# Autodesk Inventor assembly: лимонадный автомат
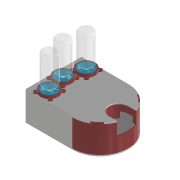
[picture p0: Inventor's stored thumbnail of the model, 180x180]
Saved by Autodesk Inventor 2022 (Build 260153000, 153)
## iProperties
Created: 2025-01-24
Part Number: лимонадный автомат
Document SubType Name: Assembly
Designer: Ivan
Author: Ivan
## Documents named in this file (8)
- E:\ВСЕ ДЕТАЛИ\лимонадный автомат.iam
- Лимонадный автомат_.iam
- E:\shoter4\Корпус.iam
- E:\shoter4\Основание верхнее.ipt
- E:\shoter4\Поворотный_модуль.iam
- E:\shoter4\Pump_V4.iam
- E:\shoter4\Держатель.ipt
- E:\ВСЕ ДЕТАЛИ\узел бутылки.iam
## Components (12 placed, 6 different names)
1. Корпус:1 [sub-assembly] — Совмещение:1, Заподлицо:1, Заподлицо:2, Совмещение:2, Совмещение:12, Совмещение:13, Совмещение:22, Совмещение:23, Совмещение:24, Совмещение:25, Совмещение:26, Совмещение:27, Совмещение:30, Совмещение:31, Совмещение:32
2. Основание верхнее:1 — Совмещение:1, Заподлицо:1, Заподлицо:2, Совмещение:2, Совмещение:33, Совмещение:34, Совмещение:35, Совмещение:36, Совмещение:37, Совмещение:38
3. Поворотный_модуль:1 [sub-assembly] — Совмещение:12, Совмещение:13
4. Pump_V4:3 [sub-assembly] — Заподлицо:5, Совмещение:18, Совмещение:19
5. Pump_V4:4 [sub-assembly] — Заподлицо:6, Совмещение:20, Совмещение:21
6. Держатель:1 — Заподлицо:5, Совмещение:18, Совмещение:19, Совмещение:22, Совмещение:24, Совмещение:25
7. Держатель:2 — Заподлицо:6, Совмещение:20, Совмещение:21, Совмещение:23, Совмещение:26, Совмещение:27
8. Держатель:3 — Совмещение:28, Заподлицо:7, Совмещение:29, Совмещение:30, Совмещение:31, Совмещение:32
9. Pump_V4:5 [sub-assembly] — Совмещение:28, Заподлицо:7, Совмещение:29
10. узел бутылки:1 [sub-assembly] — Совмещение:34, Совмещение:38
11. узел бутылки:2 [sub-assembly] — Совмещение:33, Совмещение:37
12. узел бутылки:3 [sub-assembly] — Совмещение:35, Совмещение:36
## Relationships (30: Mate 25, Flush 5)
- Совмещение:1 [Mate]: Корпус:1 ↔ Основание верхнее:1
- Заподлицо:1 [Flush]: Корпус:1 ↔ Основание верхнее:1
- Заподлицо:2 [Flush]: Корпус:1 ↔ Основание верхнее:1
- Совмещение:2 [Mate]: Корпус:1 ↔ Основание верхнее:1
- Совмещение:12 [Mate]: Корпус:1 ↔ Поворотный_модуль:1
- Совмещение:13 [Mate]: Корпус:1 ↔ Поворотный_модуль:1
- Заподлицо:5 [Flush]: Pump_V4:3 ↔ Держатель:1
- Заподлицо:6 [Flush]: Pump_V4:4 ↔ Держатель:2
- Совмещение:18 [Mate]: Pump_V4:3 ↔ Держатель:1
- Совмещение:19 [Mate]: Pump_V4:3 ↔ Держатель:1
- Совмещение:20 [Mate]: Pump_V4:4 ↔ Держатель:2
- Совмещение:21 [Mate]: Pump_V4:4 ↔ Держатель:2
- Совмещение:22 [Mate]: Корпус:1 ↔ Держатель:1
- Совмещение:23 [Mate]: Корпус:1 ↔ Держатель:2
- Совмещение:24 [Mate]: Корпус:1 ↔ Держатель:1
- Совмещение:25 [Mate]: Корпус:1 ↔ Держатель:1
- Совмещение:26 [Mate]: Корпус:1 ↔ Держатель:2
- Совмещение:27 [Mate]: Корпус:1 ↔ Держатель:2
- Совмещение:28 [Mate]: Держатель:3 ↔ Pump_V4:5
- Заподлицо:7 [Flush]: Держатель:3 ↔ Pump_V4:5
- Совмещение:29 [Mate]: Держатель:3 ↔ Pump_V4:5
- Совмещение:30 [Mate]: Корпус:1 ↔ Держатель:3
- Совмещение:31 [Mate]: Корпус:1 ↔ Держатель:3
- Совмещение:32 [Mate]: Корпус:1 ↔ Держатель:3
- Совмещение:33 [Mate]: Основание верхнее:1 ↔ узел бутылки:2
- Совмещение:34 [Mate]: Основание верхнее:1 ↔ узел бутылки:1
- Совмещение:35 [Mate]: Основание верхнее:1 ↔ узел бутылки:3
- Совмещение:36 [Mate]: Основание верхнее:1 ↔ узел бутылки:3
- Совмещение:37 [Mate]: Основание верхнее:1 ↔ узел бутылки:2
- Совмещение:38 [Mate]: Основание верхнее:1 ↔ узел бутылки:1
